# Autodesk Inventor assembly: lego human
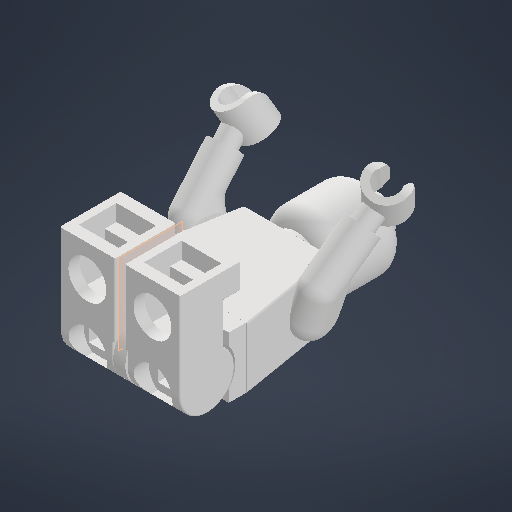
[picture p0: Inventor's stored thumbnail of the model, 512x512]
Saved by Autodesk Inventor 2027.1 (Build 311270010, 270A)
## iProperties
Created: 2026-08-07
Part Number: lego human
Document SubType Name: Assembly
Designer: lkh06
Author: lkh06
## Documents named in this file (8)
- C:\Users\lkh06\OneDrive\Desktop\Robit_HW_Design\Day2\Day02_Task07\lego human.iam
- C:\Users\lkh06\OneDrive\Desktop\Robit_HW_Design\Day2\Day02_Task07\lego arm mirrored.ipt
- C:\Users\lkh06\OneDrive\Desktop\Robit_HW_Design\Day2\Day02_Task07\Lego arm.ipt
- C:\Users\lkh06\OneDrive\Desktop\Robit_HW_Design\Day2\Day02_Task07\Lego body.ipt
- C:\Users\lkh06\OneDrive\Desktop\Robit_HW_Design\Day2\Day02_Task07\Lego connector piece.ipt
- C:\Users\lkh06\OneDrive\Desktop\Robit_HW_Design\Day2\Day02_Task07\Lego hand.ipt
- C:\Users\lkh06\OneDrive\Desktop\Robit_HW_Design\Day2\Day02_Task07\Lego head.ipt
- C:\Users\lkh06\OneDrive\Desktop\Robit_HW_Design\Day2\Day02_Task07\Lego leg.ipt
## Components (8 placed, 7 different names)
1. lego arm mirrored:1 — 회전:2, 회전:4
2. Lego arm:1 — 회전:3, 회전:5
3. Lego body:1 — 회전:1, 강체:1, 회전:2, 회전:3
4. Lego connector piece:1 — 강체:1, 회전:6
5. Lego hand:1 — 회전:4
6. Lego head:1 — 회전:1
7. Lego leg:1 — 회전:6
8. Lego hand:2 — 회전:5
## Relationships (7: RevoluteJoint 6, WeldJoint 1)
- 회전:1 [RevoluteJoint]: Lego body:1 ↔ Lego head:1
- 강체:1 [WeldJoint]: Lego body:1 ↔ Lego connector piece:1
- 회전:2 [RevoluteJoint]: lego arm mirrored:1 ↔ Lego body:1
- 회전:3 [RevoluteJoint]: Lego arm:1 ↔ Lego body:1
- 회전:4 [RevoluteJoint]: lego arm mirrored:1 ↔ Lego hand:1
- 회전:5 [RevoluteJoint]: Lego arm:1 ↔ Lego hand:2
- 회전:6 [RevoluteJoint]: Lego connector piece:1 ↔ Lego leg:1
